# Autodesk Inventor assembly: BodyStructure
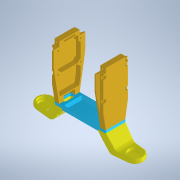
[picture p0: Inventor's stored thumbnail of the model, 180x180]
Saved by Autodesk Inventor 2022.2 (Build 262287000, 287)
## iProperties
Created: 2022-01-14
Part Number: BodyStructure
Document SubType Name: Assembly
Designer: Jochen
Author: Jochen
## Documents named in this file (4)
- D:\Projects\Chewbacca\CAD\BodyStructure.iam
- D:\Projects\Chewbacca\CAD\Body\BodyStructure Side.ipt
- D:\Projects\Chewbacca\CAD\Body\BodyStructure HipSupport.ipt
- D:\Projects\Chewbacca\CAD\Body\BodyStructure Front.ipt
## Components (5 placed, 3 different names)
1. BodyStructure Side:1 — Mate:7, Mate:8
2. BodyStructure Side:2 — Mate:5, Mate:6
3. BodyHipSupport:1 — Mate:3, Mate:4
4. BodyHipSupport:2 — Mate:1, Mate:2
5. BodyStructure Front:1 — Mate:1, Mate:2, Mate:3, Mate:4, Mate:5, Mate:6, Mate:7, Mate:8
## Relationships (8: Mate 8)
- Mate:1: BodyHipSupport:2 ↔ BodyStructure Front:1
- Mate:2: BodyHipSupport:2 ↔ BodyStructure Front:1
- Mate:3: BodyHipSupport:1 ↔ BodyStructure Front:1
- Mate:4: BodyHipSupport:1 ↔ BodyStructure Front:1
- Mate:5: BodyStructure Side:2 ↔ BodyStructure Front:1
- Mate:6: BodyStructure Side:2 ↔ BodyStructure Front:1
- Mate:7: BodyStructure Side:1 ↔ BodyStructure Front:1
- Mate:8: BodyStructure Side:1 ↔ BodyStructure Front:1
